# Autodesk Inventor assembly: link9_SubAssembly.ipt
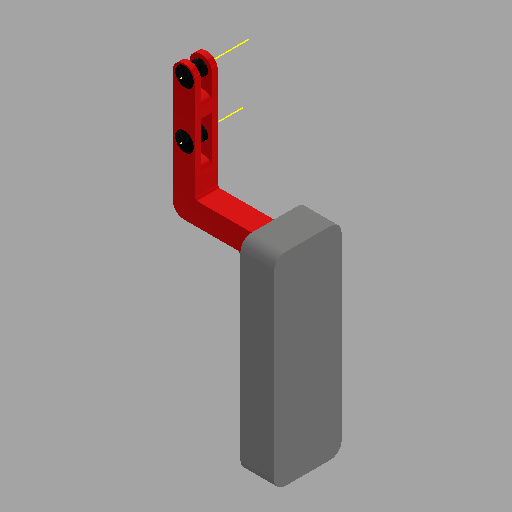
[picture p0: Inventor's stored thumbnail of the model, 512x512]
Saved by Autodesk Inventor 2024.1 (Build 281209000, 209)
## iProperties
Created: 2023-11-11
Part Number: link9_SubAssembly.ipt
Document SubType Name: Assembly
Designer: Camilo
Mass: 9.31414 g
Surface Area: 28.517 cm^2
Volume: 3.44968 cm^3
Density: 2.7 g/cm^3
Author: Camilo
## Documents named in this file (4)
- D:\Documentos\MEGA\Universidad\2023-2\DinamicaComputacionalDeSistemasMulticuerpo\DinamicaComputacionalSistemasMulticuerpo\Proyecto\CAD\3D\link10_SubAssembly.iam
- D:\Documentos\MEGA\Universidad\2023-2\DinamicaComputacionalDeSistemasMulticuerpo\DinamicaComputacionalSistemasMulticuerpo\Proyecto\CAD\3D\link10.ipt
- D:\Documentos\MEGA\Universidad\2023-2\DinamicaComputacionalDeSistemasMulticuerpo\DinamicaComputacionalSistemasMulticuerpo\Proyecto\CAD\3D\bolt.ipt
- D:\Documentos\MEGA\Universidad\2023-2\DinamicaComputacionalDeSistemasMulticuerpo\DinamicaComputacionalSistemasMulticuerpo\Proyecto\CAD\3D\jaw.ipt
## Components (6 placed, 3 different names)
1. link10:1 — Insert:1, Insert:2, Insert:3, Insert:4, Mate:1
2. bolt:1 — Insert:1
3. bolt:2 — Insert:2
4. bolt:3 — Insert:3
5. bolt:4 — Insert:4
6. jaw:1 — Mate:1
## Relationships (5: Insert 4, Mate 1)
- Insert:1: link10:1 ↔ bolt:1
- Insert:2: link10:1 ↔ bolt:2
- Insert:3: link10:1 ↔ bolt:3
- Insert:4: link10:1 ↔ bolt:4
- Mate:1: link10:1 ↔ jaw:1
